# Autodesk Inventor assembly: torch_light_injection_assembly_v0-1_20feb25.ipt
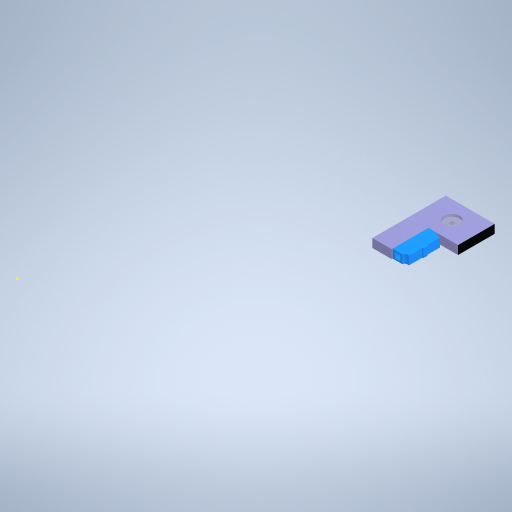
[picture p0: Inventor's stored thumbnail of the model, 512x512]
Saved by Autodesk Inventor 2024 (Build 280153000, 153)
## iProperties
Created: 2025-02-20
Part Number: torch_light_injection_assembly_v0-1_20feb25.ipt
Document SubType Name: Assembly
Designer: phdgc
Author: phdgc
## Documents named in this file (5)
- C:\Users\phdgc\OneDrive - University of Bristol\TORCH\Light Injection\torch_light_injection_assembly_v0-1_20feb25.ipt.iam
- C:\Users\phdgc\OneDrive - University of Bristol\TORCH\Light Injection\torch_light_injection_3d_pirnt_v0-1_20feb25.ipt
- C:\Users\phdgc\OneDrive - University of Bristol\TORCH\Light Injection\lc_lc_coupler_molex_1061251100_sd_scaled_3d.ipt
- C:\Users\phdgc\OneDrive - University of Bristol\TORCH\Light Injection\MRA03-E02-Prism_Mirror.ipt
- C:\Users\phdgc\OneDrive - University of Bristol\TORCH\Light Injection\DG05-220-Diffuser.ipt
## Components (4 placed, 4 different names)
1. torch_light_injection_3d_pirnt_v0-1_20feb25:1 — Mate:1, Mate:2, Flush:1, Mate:3, Mate:4, Mate:5, Insert:1
2. lc_lc_coupler_molex_1061251100_sd_scaled_3d:1 — Mate:1, Mate:2, Flush:1
3. MRA03-E02-Prism_Mirror:1 — Mate:3, Mate:4, Mate:5
4. DG05-220-Diffuser:1 — Insert:1
## Relationships (7: Mate 5, Flush 1, Insert 1)
- Mate:1: torch_light_injection_3d_pirnt_v0-1_20feb25:1 ↔ lc_lc_coupler_molex_1061251100_sd_scaled_3d:1
- Mate:2: torch_light_injection_3d_pirnt_v0-1_20feb25:1 ↔ lc_lc_coupler_molex_1061251100_sd_scaled_3d:1
- Flush:1: torch_light_injection_3d_pirnt_v0-1_20feb25:1 ↔ lc_lc_coupler_molex_1061251100_sd_scaled_3d:1
- Mate:3: torch_light_injection_3d_pirnt_v0-1_20feb25:1 ↔ MRA03-E02-Prism_Mirror:1
- Mate:4: torch_light_injection_3d_pirnt_v0-1_20feb25:1 ↔ MRA03-E02-Prism_Mirror:1
- Mate:5: torch_light_injection_3d_pirnt_v0-1_20feb25:1 ↔ MRA03-E02-Prism_Mirror:1
- Insert:1 (-1.5 mm): torch_light_injection_3d_pirnt_v0-1_20feb25:1 ↔ DG05-220-Diffuser:1
## Named parameters: Finish1_Area = 21.6172
note: some values were not read from the file. Shown as the stored number, unit unknown: "Finish1_Area".
